# Autodesk Inventor assembly: Assembly1
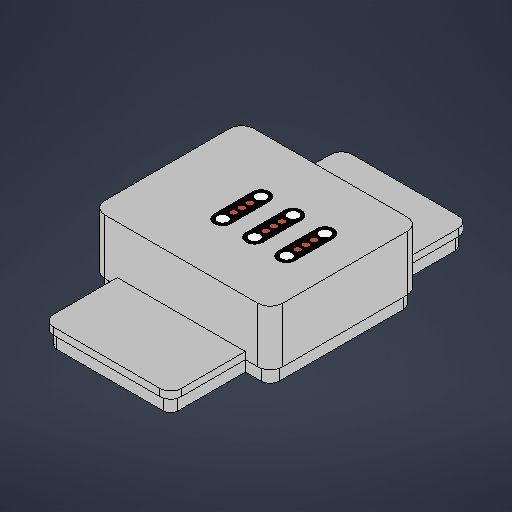
[picture p0: Inventor's stored thumbnail of the model, 512x512]
Saved by Autodesk Inventor 2026 (Build 300175000, 175)
## iProperties
Created: 2025-04-14
Part Number: Assembly1
Document SubType Name: Assembly
Designer: ct_vi
Author: ct_vi
## Documents named in this file (3)
- C:\Users\ct_vi\Documents\Capstone_Research_3D_Files\Assembly1.iam
- C:\Users\ct_vi\Documents\Capstone_Research_3D_Files\Body_Up.ipt
- C:\Users\ct_vi\Documents\Capstone_Research_3D_Files\Pogo_Set1.iam
## Components (4 placed, 2 different names)
1. Body_Up:1 — Mate:1, Mate:2, Flush:1, Mate:3, Mate:4, Flush:2, Mate:5, Mate:6, Flush:3
2. Pogo_Set1:1 [sub-assembly] — Mate:5, Mate:6, Flush:3
3. Pogo_Set1:2 [sub-assembly] — Mate:1, Mate:2, Flush:1
4. Pogo_Set1:3 [sub-assembly] — Mate:3, Mate:4, Flush:2
## Relationships (9: Mate 6, Flush 3)
- Mate:1: Body_Up:1 ↔ Pogo_Set1:2
- Mate:2: Body_Up:1 ↔ Pogo_Set1:2
- Flush:1: Body_Up:1 ↔ Pogo_Set1:2
- Mate:3: Body_Up:1 ↔ Pogo_Set1:3
- Mate:4: Body_Up:1 ↔ Pogo_Set1:3
- Flush:2: Body_Up:1 ↔ Pogo_Set1:3
- Mate:5: Body_Up:1 ↔ Pogo_Set1:1
- Mate:6: Body_Up:1 ↔ Pogo_Set1:1
- Flush:3: Body_Up:1 ↔ Pogo_Set1:1
